# Autodesk Inventor assembly: wall_54_assembly
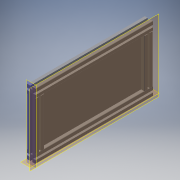
[picture p0: Inventor's stored thumbnail of the model, 180x180]
Saved by Autodesk Inventor 2016 (Build 200138000, 138)
## iProperties
Created: 2015-09-04
Part Number: wall_54_assembly
Document SubType Name: Assembly
Designer: oscar
Author: oscar
## Documents named in this file (4)
- C:\Users\oscar\Desktop\rockin_parts\wall_54\inventor\wall_54_assembly.iam
- C:\Users\oscar\Desktop\rockin_parts\wall_54\inventor\B4040_220.ipt
- C:\Users\oscar\Desktop\rockin_parts\wall_54\inventor\B4040_540.ipt
- C:\Users\oscar\Desktop\rockin_parts\wall_54\inventor\wall.ipt
## Components (5 placed, 3 different names)
1. B4040_220:1 — Mate:1, Flush:1, Flush:2, Mate:3, Flush:4, Flush:5, Mate:4, Mate:7
2. B4040_220:2 — Mate:2, Flush:3, Flush:6
3. B4040_540:1 — Mate:1, Flush:1, Flush:2, Mate:2, Flush:3, Flush:7, Mate:5, Mate:6, Flush:8
4. B4040_540:2 — Mate:3, Flush:4, Flush:5, Flush:6
5. wall:1 — Flush:7, Mate:4, Mate:5
## Relationships (15: Flush 8, Mate 7)
- Mate:1: B4040_220:1 ↔ B4040_540:1
- Flush:1: B4040_220:1 ↔ B4040_540:1
- Flush:2: B4040_220:1 ↔ B4040_540:1
- Mate:2: B4040_220:2 ↔ B4040_540:1
- Flush:3: B4040_220:2 ↔ B4040_540:1
- Mate:3: B4040_220:1 ↔ B4040_540:2
- Flush:4: B4040_220:1 ↔ B4040_540:2
- Flush:5: B4040_220:1 ↔ B4040_540:2
- Flush:6: B4040_220:2 ↔ B4040_540:2
- Flush:7 (17.5 mm): B4040_540:1 ↔ wall:1
- Mate:4: B4040_220:1 ↔ wall:1
- Mate:5: B4040_540:1 ↔ wall:1
- Mate:6: B4040_540:1
- Flush:8: B4040_540:1
- Mate:7: B4040_220:1
